# Autodesk Inventor assembly: VP Input to 2X Ring Gears to 90 Degree to VP Output
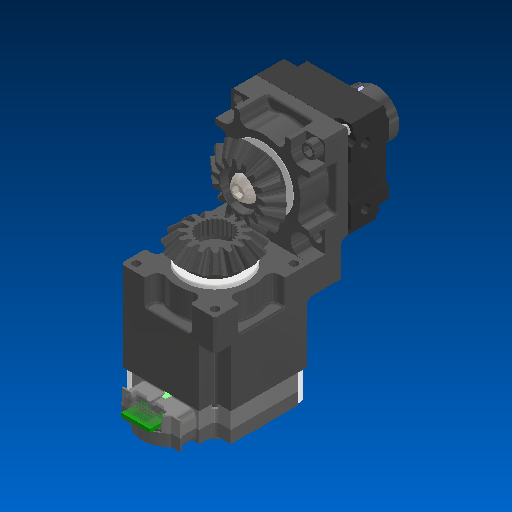
[picture p0: Inventor's stored thumbnail of the model, 512x512]
Saved by Autodesk Inventor 2022.2 (Build 262287000, 287)
## iProperties
Created: 2018-09-07
Part Number: VP Input to 2X Ring Gears to 90 Degree to VP Output
Description: STEP AP214
Document SubType Name: Assembly
Designer: omard
Mass: 195.44 g
Surface Area: 1051.92 cm^2
Volume: 139.105 cm^3
Density: 1.40498 g/cm^3
Sending System: SolidWorks 2017
Preprocessor: SwSTEP 2.0
Title: VP Input to 2X Ring Gears to 90 Degree to VP Output.STEP
Revision Number: ANY
## Documents named in this file (10)
- D:\omard\OneDrive - Auburn University\BasketBall Shooting Robot\VEX Parts\VP Input to 2X Ring Gears to 90 Degree to VP Output.iam
- D:\omard\OneDrive - Auburn University\BasketBall Shooting Robot\VEX Parts\Components\217-6293-000 Rev1.iam
- D:\omard\OneDrive - Auburn University\BasketBall Shooting Robot\VEX Parts\Components\VersaPlanetary Output Blocks_VP Output Block.iam
- D:\omard\OneDrive - Auburn University\BasketBall Shooting Robot\VEX Parts\Components\VersaPlanetary Ring Gears_VP Ring Gear.iam
- D:\omard\OneDrive - Auburn University\BasketBall Shooting Robot\VEX Parts\Components\217-2816-001 Rev1.ipt
- D:\omard\OneDrive - Auburn University\BasketBall Shooting Robot\VEX Parts\Components\VersaPlanetary Gear Sets_10_1 (217-2820).iam
- D:\omard\OneDrive - Auburn University\BasketBall Shooting Robot\VEX Parts\Components\217-2820-000 Rev2_Public.iam
- D:\omard\OneDrive - Auburn University\BasketBall Shooting Robot\VEX Parts\Components\#8-32 SHCS, Grade 8 Steel Rev2_SSA0832-0875ZB.ipt
- D:\omard\OneDrive - Auburn University\BasketBall Shooting Robot\VEX Parts\Universal Female Output Shaft 1_2 Hex.iam
- D:\omard\OneDrive - Auburn University\BasketBall Shooting Robot\VEX Parts\VersaPlanetary Integrated Encoder (217-5046).iam
## Components (10 placed, 10 different names)
1. 217-6293-000 Rev1_1 [sub-assembly] — Mate:2, Angle:1, Mate:8, Angle:2, Mate:14, Mate:15, Angle:3
2. VersaPlanetary Output Blocks_VP Output Block_3 [sub-assembly] — Mate:1, Mate:8, Angle:2, Angle:3
3. VersaPlanetary Ring Gears_VP Ring Gear_5 [sub-assembly] — Mate:10, Mate:11, Mate:12, Mate:15
4. 217-2816-001 Rev1_6 — Mate:3, Mate:5, Mate:7, Mate:9, Mate:12
5. VersaPlanetary Gear Sets_10:1 (217-2820)_7 [sub-assembly]
6. 217-2820-000 Rev2_Public_8 [sub-assembly] — Mate:6
7. #8-32 SHCS, Grade 8 Steel Rev2_SSA0832-0875ZB_10
8. #8-32 SHCS, Grade 8 Steel Rev2_SSA0832-0875ZB_11
9. Universal Female Output Shaft 1_2 Hex:1 [sub-assembly] — Mate:1, Mate:2
10. VersaPlanetary Integrated Encoder (217-5046):1 [sub-assembly] — Mate:3, Mate:5, Angle:1, Mate:6, Mate:7, Mate:9, Mate:10, Mate:11, Mate:14
## Relationships (16: Mate 13, Angle 3)
- Mate:1: VersaPlanetary Output Blocks_VP Output Block_3 ↔ Universal Female Output Shaft 1_2 Hex:1
- Mate:2: 217-6293-000 Rev1_1 ↔ Universal Female Output Shaft 1_2 Hex:1
- Mate:3: 217-2816-001 Rev1_6 ↔ VersaPlanetary Integrated Encoder (217-5046):1
- Mate:5: 217-2816-001 Rev1_6 ↔ VersaPlanetary Integrated Encoder (217-5046):1
- Angle:1 (0 deg): 217-6293-000 Rev1_1 ↔ VersaPlanetary Integrated Encoder (217-5046):1
- Mate:6: 217-2820-000 Rev2_Public_8 ↔ VersaPlanetary Integrated Encoder (217-5046):1
- Mate:7: 217-2816-001 Rev1_6 ↔ VersaPlanetary Integrated Encoder (217-5046):1
- Mate:8: 217-6293-000 Rev1_1 ↔ VersaPlanetary Output Blocks_VP Output Block_3
- Angle:2 (0 deg): 217-6293-000 Rev1_1 ↔ VersaPlanetary Output Blocks_VP Output Block_3
- Mate:9: 217-2816-001 Rev1_6 ↔ VersaPlanetary Integrated Encoder (217-5046):1
- Mate:10: VersaPlanetary Ring Gears_VP Ring Gear_5 ↔ VersaPlanetary Integrated Encoder (217-5046):1
- Mate:11: VersaPlanetary Ring Gears_VP Ring Gear_5 ↔ VersaPlanetary Integrated Encoder (217-5046):1
- Mate:12: VersaPlanetary Ring Gears_VP Ring Gear_5 ↔ 217-2816-001 Rev1_6
- Mate:14: 217-6293-000 Rev1_1 ↔ VersaPlanetary Integrated Encoder (217-5046):1
- Mate:15: 217-6293-000 Rev1_1 ↔ VersaPlanetary Ring Gears_VP Ring Gear_5
- Angle:3 (0 deg): 217-6293-000 Rev1_1 ↔ VersaPlanetary Output Blocks_VP Output Block_3
